# Autodesk Inventor assembly: maniac
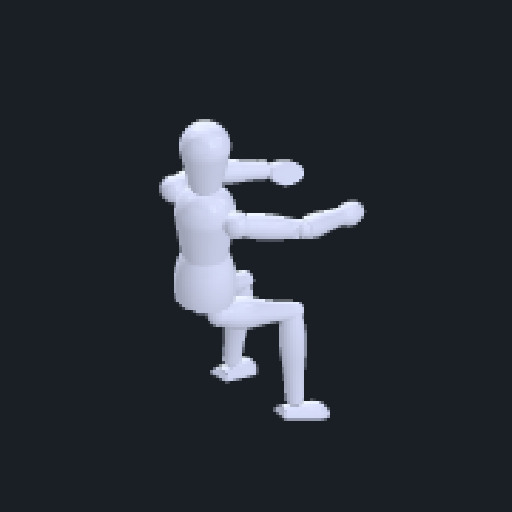
[picture p0: Inventor's stored thumbnail of the model, 512x512]
Saved by Autodesk Inventor 2025.3 (Build 293356000, 356)
## iProperties
Created: 2026-08-12
Part Number: maniac
Document SubType Name: Assembly
Designer: VianaCC
Author: VianaCC
## Documents named in this file (12)
- C:\Users\vianacc\Documents\GitHub\utv_startup\products\utv\ergonomics\cad\reference\maniac.iam
- C:\Users\vianacc\Documents\GitHub\utv_startup\products\utv\ergonomics\cad\reference\parts\Arm.ipt
- C:\Users\vianacc\Documents\GitHub\utv_startup\products\utv\ergonomics\cad\reference\parts\Body.ipt
- C:\Users\vianacc\Documents\GitHub\utv_startup\products\utv\ergonomics\cad\reference\parts\Femur.ipt
- C:\Users\vianacc\Documents\GitHub\utv_startup\products\utv\ergonomics\cad\reference\parts\Foot.ipt
- C:\Users\vianacc\Documents\GitHub\utv_startup\products\utv\ergonomics\cad\reference\parts\Forearm.ipt
- C:\Users\vianacc\Documents\GitHub\utv_startup\products\utv\ergonomics\cad\reference\parts\Hand.ipt
- C:\Users\vianacc\Documents\GitHub\utv_startup\products\utv\ergonomics\cad\reference\parts\Head.ipt
- C:\Users\vianacc\Documents\GitHub\utv_startup\products\utv\ergonomics\cad\reference\parts\Hip.ipt
- C:\Users\vianacc\Documents\GitHub\utv_startup\products\utv\ergonomics\cad\reference\parts\Pelvis.ipt
- C:\Users\vianacc\Documents\GitHub\utv_startup\products\utv\ergonomics\cad\reference\parts\Sura.ipt
- C:\Users\vianacc\Documents\GitHub\utv_startup\products\utv\ergonomics\cad\reference\parts\Waist.ipt
## Components (18 placed, 11 different names)
1. Head:1 — Mate:1, Flush:1, Angle:1
2. Body:1 — Mate:1, Mate:2, Mate:5, Mate:13, Flush:1, Angle:1, Mate:19, Angle:21, Angle:32, Angle:33, Angle:38, Angle:39
3. Pelvis:1 — Mate:6, Mate:7, Mate:17, Mate:19, Angle:21, Angle:22, Angle:23, Angle:24, Angle:25, Mate:20
4. Waist:1 — Mate:5, Mate:6
5. Arm:1 — Mate:2, Mate:3, Angle:32, Angle:33, Angle:34, Angle:35
6. Forearm:1 — Mate:3, Mate:4, Angle:34, Angle:35, Angle:36, Angle:37
7. Hand:1 — Mate:4, Angle:36, Angle:37
8. Arm:2 — Mate:13, Angle:38, Angle:39, Angle:40, Angle:41
9. Forearm:2 — Angle:40, Angle:41, Angle:42, Angle:43
10. Hand:2 — Angle:42, Angle:43
11. Femur:1 — Mate:9, Mate:18, Angle:22, Angle:23, Angle:26, Mate:21, Angle:28
12. Foot:1 — Mate:10, Angle:27, Angle:28
13. Hip:1 — Mate:7, Mate:18
14. Sura:1 — Mate:9, Mate:10, Angle:26, Mate:21, Angle:27
15. Femur:2 — Angle:24, Angle:25, Mate:22, Angle:29
16. Foot:2 — Angle:30, Angle:31
17. Hip:2 — Mate:17
18. Sura:2 — Mate:22, Angle:29, Angle:30, Angle:31
## Relationships (46: Angle 24, Mate 21, Flush 1)
- Mate:1: Head:1 ↔ Body:1
- Mate:2: Body:1 ↔ Arm:1
- Mate:3: Arm:1 ↔ Forearm:1
- Mate:4: Forearm:1 ↔ Hand:1
- Mate:5: Body:1 ↔ Waist:1
- Mate:6: Pelvis:1 ↔ Waist:1
- Mate:7: Pelvis:1 ↔ Hip:1
- Mate:9: Femur:1 ↔ Sura:1
- Mate:10: Foot:1 ↔ Sura:1
- [Mate]: Arm:2 ↔ Forearm:2
- [Mate]: Forearm:2 ↔ Hand:2
- Mate:13: Body:1 ↔ Arm:2
- [Mate]: Femur:2 ↔ Hip:2
- [Mate]: Femur:2 ↔ Sura:2
- [Mate]: Foot:2 ↔ Sura:2
- Mate:17: Pelvis:1 ↔ Hip:2
- Mate:18: Femur:1 ↔ Hip:1
- Flush:1: Head:1 ↔ Body:1
- Angle:1 (0 deg): Head:1 ↔ Body:1
- Mate:19: Body:1 ↔ Pelvis:1
- Angle:21 (180 deg): Body:1 ↔ Pelvis:1
- Angle:22 (10 deg): Pelvis:1 ↔ Femur:1
- Angle:23 (80 deg): Pelvis:1 ↔ Femur:1
- Angle:24 (-80 deg): Pelvis:1 ↔ Femur:2
- Angle:25 (10 deg): Pelvis:1 ↔ Femur:2
- Mate:20: Pelvis:1
- Angle:26 (-40 deg): Femur:1 ↔ Sura:1
- Mate:21: Femur:1 ↔ Sura:1
- Angle:27 (160 deg): Foot:1 ↔ Sura:1
- Angle:28 (0 deg): Femur:1 ↔ Foot:1
- Mate:22: Femur:2 ↔ Sura:2
- Angle:29 (-40 deg): Femur:2 ↔ Sura:2
- Angle:30 (180 deg): Foot:2 ↔ Sura:2
- Angle:31 (20 deg): Foot:2 ↔ Sura:2
- Angle:32 (200 deg): Body:1 ↔ Arm:1
- Angle:33 (160 deg): Body:1 ↔ Arm:1
- Angle:34 (0 deg): Arm:1 ↔ Forearm:1
- Angle:35 (-40 deg): Arm:1 ↔ Forearm:1
- Angle:36 (-90 deg): Forearm:1 ↔ Hand:1
- Angle:37 (-15 deg): Forearm:1 ↔ Hand:1
- Angle:38 (-20 deg): Body:1 ↔ Arm:2
- Angle:39 (20 deg): Body:1 ↔ Arm:2
- Angle:40 (0 deg): Arm:2 ↔ Forearm:2
- Angle:41 (-30 deg): Arm:2 ↔ Forearm:2
- Angle:42 (180 deg): Forearm:2 ↔ Hand:2
- Angle:43 (0 deg): Forearm:2 ↔ Hand:2
## Named parameters: d10_d2 = 0 mm, d11_d3 = 0 mm, d13_d7 = 0 mm, d14_d8 = 0 mm, d15_d9 = 0 mm, headbody = 0 deg, bodypelvis = 180 deg, right_elbow = -30 deg, right_wrist = 0 deg
